# Autodesk Inventor assembly: INA260_with_pins
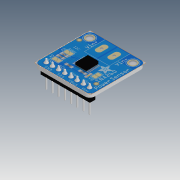
[picture p0: Inventor's stored thumbnail of the model, 180x180]
Saved by Autodesk Inventor 2020 (Build 240168000, 168)
## iProperties
Created: 2020-09-27
Part Number: INA260_with_pins
Document SubType Name: Assembly
Designer: DELL
Author: DELL
## Documents named in this file (3)
- F:\SoftRobot\Model\FlexipodHardware-master\mechanical_model\Adafruit_INA260\INA260_with_pins.iam
- F:\SoftRobot\Model\FlexipodHardware-master\mechanical_model\Adafruit_INA260\Adafruit_INA260.ipt
- F:\SoftRobot\Model\FlexipodHardware-master\mechanical_model\pins.ipt
## Components (9 placed, 2 different names)
1. Adafruit_INA260:1 — Mate:1, Mate:2, Angle:1
2. pins:1 — Mate:1, Mate:2, Angle:1
3. pins:2
4. pins:3
5. pins:4
6. pins:5
7. pins:6
8. pins:7
9. pins:8
## Component patterns: (8 elements, first: pins:1)
## Relationships (3: Mate 2, Angle 1)
- Mate:1: Adafruit_INA260:1 ↔ pins:1
- Mate:2: Adafruit_INA260:1 ↔ pins:1
- Angle:1 (0 deg): Adafruit_INA260:1 ↔ pins:1
